# Autodesk Inventor assembly: モーター1：1
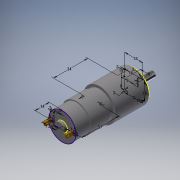
[picture p0: Inventor's stored thumbnail of the model, 180x180]
Saved by Autodesk Inventor 2018 (Build 220112000, 112)
## iProperties
Part Number: モーター1：1
Material: 一般
Document SubType Name: Assembly
Designer: eieio
Author: eieio
## Documents named in this file (4)
- C:\Users\eieio\Documents\CAD\メカナムロボット\モーター100：1.iam
- C:\Users\eieio\Documents\CAD\メカナムロボット\モーター100：1.ipt
- C:\Users\eieio\Documents\CAD\交ロボ\モーター端子.ipt
- C:\Users\eieio\Documents\CAD\メカナムロボット\モーター100：1軸.ipt
## Components (4 placed, 3 different names)
1. モーター100：1:1 — メイト:1, メイト:2, メイト:3, メイト:4, メイト:5, メイト:6, 挿入:1
2. モーター端子:1 — メイト:1, メイト:5, メイト:6
3. モーター端子:2 — メイト:2, メイト:3, メイト:4
4. モーター100：1軸:1 — 挿入:1
## Relationships (7: Mate 6, Insert 1)
- メイト:1 [Mate]: モーター100：1:1 ↔ モーター端子:1
- メイト:2 [Mate]: モーター100：1:1 ↔ モーター端子:2
- メイト:3 [Mate]: モーター100：1:1 ↔ モーター端子:2
- メイト:4 [Mate]: モーター100：1:1 ↔ モーター端子:2
- メイト:5 [Mate]: モーター100：1:1 ↔ モーター端子:1
- メイト:6 [Mate]: モーター100：1:1 ↔ モーター端子:1
- 挿入:1 [Insert]: モーター100：1:1 ↔ モーター100：1軸:1
